# Autodesk Inventor assembly: VER2.0_MIR_CPY_MIR_MIR
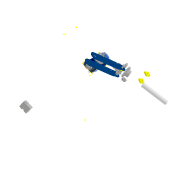
[picture p0: Inventor's stored thumbnail of the model, 180x180]
Saved by Autodesk Inventor 2020.5 (Build 245400000, 400)
## iProperties
Created: 2022-10-31
Part Number: VER2.0_MIR_CPY_MIR_MIR
Document SubType Name: Assembly
Designer: Administrator
Author: Administrator
## Documents named in this file (18)
- C:\Users\Administrator\Documents\kamuy2\kamuy2\VER2.0_MIR_CPY_MIR_MIR.iam
- C:\Users\Administrator\Documents\kamuy2\kamuy2\Parts\Part2_MIR_CPY_MIR_MIR.ipt
- C:\Users\Administrator\Documents\kamuy2\kamuy2\Parts\x-540_idle_MIR_CPY_MIR_MIR.ipt
- C:\Users\Administrator\Documents\kamuy2\kamuy2\Parts\GEABP1.0-32-10-A-12-KFC22-K3_Autodesk_Inventor_2020_20221101\AIS2020\GEABP1_0-32-10-A-12-KFC22-K3_MIR_CPY_MIR_MIR.iam
- C:\Users\Administrator\Documents\kamuy2\kamuy2\Parts\GEYK1.0-70-10-B-10K_Autodesk_Inventor_2020_20221114\AIS2020\GEYK1_0-70-10-B-10K_MIR_CPY_MIR_MIR.iam
- C:\Users\Administrator\Documents\kamuy2\kamuy2\Part16_MIR_CPY_MIR_MIR.ipt
- C:\Users\Administrator\Documents\kamuy2\kamuy2\Part1_MIR_CPY_MIR_MIR.ipt
- C:\Users\Administrator\Documents\kamuy2\kamuy2\Part13_MIR_CPY_MIR_MIR.ipt
- C:\Users\Administrator\Documents\kamuy2\kamuy2\Part17_MIR_CPY_MIR_MIR.ipt
- C:\Users\Administrator\Documents\kamuy2\kamuy2\Parts\SMYHF10_STEP_AP203AP214\SMYHF10_203_MIR_CPY_MIR_MIR.ipt
- C:\Users\Administrator\Documents\kamuy2\kamuy2\Parts\BGHK6800VV-30_Autodesk_Inventor_2020_20221102\AIS2020\BGHK6800VV-30_MIR_CPY_MIR_MIR.iam
- C:\Users\Administrator\Documents\kamuy2\kamuy2\Parts\XW540.N105.I101_MIR_CPY_MIR_MIR.ipt
- C:\Users\Administrator\Documents\kamuy2\kamuy2\Parts\NSFMKR10-67-KA22-A20_Autodesk_Inventor_2020_20221116\AIS2020\NSFMKR10-67-KA22-A20_MIR_CPY_MIR_MIR.iam
- C:\Users\Administrator\Documents\kamuy2\kamuy2\Parts\NSFMR10-37_Autodesk_Inventor_2020_20221116\AIS2020\NSFMR10-37(000_000)_MIR_CPY_MIR_MIR.iam
- C:\Users\Administrator\Documents\kamuy2\kamuy2\Parts\NSFMKRRA10-144-F3-S6-KA5-A18-KB108.5-B11_Autodesk_Inventor_2020_20221117\AIS2020\NSFMKRRA10-144-F3-S6-KA5-A18-KB108_5-B11_MIR_CPY_MIR_MIR.iam
- C:\Users\Administrator\Documents\kamuy2\kamuy2\LEG_MIR_MIR1_MIR.iam
- C:\Users\Administrator\Documents\kamuy2\kamuy2\Parts\BGTAB6900VV_Autodesk_Inventor_2020_20221121\AIS2020\BGTAB6900VV.iam
- C:\Users\Administrator\Documents\kamuy2\kamuy2\3dprinter\Part7.ipt
## Components (29 placed, 17 different names)
1. Part2_MIR_CPY_MIR_MIR:1
2. x-540_idle_MIR_CPY_MIR_MIR:1 — メイト:50, メイト:51, フラッシュ:58, フラッシュ:66, フラッシュ:68, メイト:258, メイト:154, メイト:166, フラッシュ:103, メイト:256
3. GEABP1_0-32-10-A-12-KFC22-K3_MIR_CPY_MIR_MIR:1 [sub-assembly] — メイト:50, メイト:51, フラッシュ:31
4. GEYK1_0-70-10-B-10K_MIR_CPY_MIR_MIR:1 [sub-assembly] — フラッシュ:61, メイト:248, フラッシュ:136
5. x-540_idle_MIR_CPY_MIR_MIR:2 — フラッシュ:58, フラッシュ:66, フラッシュ:68, メイト:85, メイト:86, メイト:168, フラッシュ:100, メイト:183, メイト:178, メイト:179, メイト:180
6. GEABP1_0-32-10-A-12-KFC22-K3_MIR_CPY_MIR_MIR:2 [sub-assembly] — メイト:85, メイト:86, フラッシュ:61
7. Part16_MIR_CPY_MIR_MIR:1 — メイト:258, フラッシュ:92, メイト:170
8. Part16_MIR_CPY_MIR_MIR:2 — フラッシュ:92, メイト:154, メイト:168, メイト:171, フラッシュ:141
9. Part1_MIR_CPY_MIR_MIR:1 — フラッシュ:100, メイト:171, フラッシュ:141
10. Part1_MIR_CPY_MIR_MIR:2 — メイト:166, メイト:170, メイト:183
11. Part13_MIR_CPY_MIR_MIR:1 — フラッシュ:103, メイト:172, フラッシュ:104, フラッシュ:108, メイト:208
12. Part17_MIR_CPY_MIR_MIR:1 — メイト:172, フラッシュ:104, フラッシュ:108, メイト:174, フラッシュ:105, メイト:177
13. SMYHF10_203_MIR_CPY_MIR_MIR:1 — メイト:174, フラッシュ:105, メイト:254
14. GEYK1_0-70-10-B-10K_MIR_CPY_MIR_MIR:2 [sub-assembly] — メイト:177, メイト:65, メイト:207
15. Part13_MIR_CPY_MIR_MIR:2 — メイト:178, メイト:179, メイト:180, メイト:194, フラッシュ:110, メイト:214
16. SMYHF10_203_MIR_CPY_MIR_MIR:2 — メイト:185, メイト:187, メイト:213
17. Part17_MIR_CPY_MIR_MIR:2 — メイト:185, メイト:187, メイト:194, フラッシュ:110, メイト:211, メイト:215, メイト:40
18. BGHK6800VV-30_MIR_CPY_MIR_MIR:1 [sub-assembly] — メイト:65, メイト:205, フラッシュ:32, フラッシュ:33, メイト:209, フラッシュ:115, フラッシュ:116
19. GEABP1_0-32-10-A-12-KFC22-K3_MIR_CPY_MIR_MIR:3 [sub-assembly] — メイト:203, メイト:204
20. XW540.N105.I101_MIR_CPY_MIR_MIR:1 — メイト:203, メイト:204, メイト:205, フラッシュ:32, フラッシュ:33, フラッシュ:17, メイト:42
21. NSFMKR10-67-KA22-A20_MIR_CPY_MIR_MIR:1 [sub-assembly] — メイト:207, メイト:208, メイト:209, メイト:254, メイト:41
22. BGHK6800VV-30_MIR_CPY_MIR_MIR:2 [sub-assembly] — フラッシュ:115, フラッシュ:116, メイト:211, メイト:212
23. NSFMR10-37(000_000)_MIR_CPY_MIR_MIR:1 [sub-assembly] — メイト:212, メイト:213, メイト:214, メイト:215, メイト:39
24. NSFMKRRA10-144-F3-S6-KA5-A18-KB108_5-B11_MIR_CPY_MIR_MIR:1 [sub-assembly] — メイト:248, フラッシュ:136, メイト:256, メイト:64
25. LEG_MIR_MIR1_MIR:1 [sub-assembly] — メイト:64, フラッシュ:31
26. BGTAB6900VV:1 [sub-assembly] — メイト:39, メイト:40, フラッシュ:18
27. BGTAB6900VV:2 [sub-assembly] — メイト:41, フラッシュ:17, メイト:42, フラッシュ:18
28. x-540_idle_MIR_CPY_MIR_MIR:3 — フラッシュ:19
29. Part7:1 — フラッシュ:19
## Relationships (61: Mate 42, Flush 19)
- メイト:50 [Mate] (4 mm): x-540_idle_MIR_CPY_MIR_MIR:1 ↔ GEABP1_0-32-10-A-12-KFC22-K3_MIR_CPY_MIR_MIR:1
- メイト:51 [Mate]: x-540_idle_MIR_CPY_MIR_MIR:1 ↔ GEABP1_0-32-10-A-12-KFC22-K3_MIR_CPY_MIR_MIR:1
- フラッシュ:58 [Flush]: x-540_idle_MIR_CPY_MIR_MIR:1 ↔ x-540_idle_MIR_CPY_MIR_MIR:2
- フラッシュ:66 [Flush]: x-540_idle_MIR_CPY_MIR_MIR:1 ↔ x-540_idle_MIR_CPY_MIR_MIR:2
- フラッシュ:68 [Flush]: x-540_idle_MIR_CPY_MIR_MIR:1 ↔ x-540_idle_MIR_CPY_MIR_MIR:2
- メイト:85 [Mate]: x-540_idle_MIR_CPY_MIR_MIR:2 ↔ GEABP1_0-32-10-A-12-KFC22-K3_MIR_CPY_MIR_MIR:2
- メイト:86 [Mate] (4 mm): x-540_idle_MIR_CPY_MIR_MIR:2 ↔ GEABP1_0-32-10-A-12-KFC22-K3_MIR_CPY_MIR_MIR:2
- フラッシュ:61 [Flush]: GEYK1_0-70-10-B-10K_MIR_CPY_MIR_MIR:1 ↔ GEABP1_0-32-10-A-12-KFC22-K3_MIR_CPY_MIR_MIR:2
- メイト:258 [Mate] (15.591 mm): x-540_idle_MIR_CPY_MIR_MIR:1 ↔ Part16_MIR_CPY_MIR_MIR:1
- フラッシュ:92 [Flush]: Part16_MIR_CPY_MIR_MIR:1 ↔ Part16_MIR_CPY_MIR_MIR:2
- メイト:154 [Mate] (15.591 mm): x-540_idle_MIR_CPY_MIR_MIR:1 ↔ Part16_MIR_CPY_MIR_MIR:2
- メイト:168 [Mate] (15.591 mm): x-540_idle_MIR_CPY_MIR_MIR:2 ↔ Part16_MIR_CPY_MIR_MIR:2
- フラッシュ:100 [Mate]: x-540_idle_MIR_CPY_MIR_MIR:2 ↔ Part1_MIR_CPY_MIR_MIR:1
- メイト:171 [Mate]: Part16_MIR_CPY_MIR_MIR:2 ↔ Part1_MIR_CPY_MIR_MIR:1
- フラッシュ:141 [Flush] (12.859 mm): Part16_MIR_CPY_MIR_MIR:2 ↔ Part1_MIR_CPY_MIR_MIR:1
- メイト:166 [Mate]: x-540_idle_MIR_CPY_MIR_MIR:1 ↔ Part1_MIR_CPY_MIR_MIR:2
- メイト:170 [Mate]: Part16_MIR_CPY_MIR_MIR:1 ↔ Part1_MIR_CPY_MIR_MIR:2
- メイト:183 [Mate]: x-540_idle_MIR_CPY_MIR_MIR:2 ↔ Part1_MIR_CPY_MIR_MIR:2
- フラッシュ:103 [Mate]: x-540_idle_MIR_CPY_MIR_MIR:1 ↔ Part13_MIR_CPY_MIR_MIR:1
- メイト:172 [Mate] (15 mm): Part13_MIR_CPY_MIR_MIR:1 ↔ Part17_MIR_CPY_MIR_MIR:1
- フラッシュ:104 [Flush]: Part13_MIR_CPY_MIR_MIR:1 ↔ Part17_MIR_CPY_MIR_MIR:1
- フラッシュ:108 [Flush]: Part13_MIR_CPY_MIR_MIR:1 ↔ Part17_MIR_CPY_MIR_MIR:1
- メイト:174 [Mate]: Part17_MIR_CPY_MIR_MIR:1 ↔ SMYHF10_203_MIR_CPY_MIR_MIR:1
- フラッシュ:105 [Flush] (0.1 mm): Part17_MIR_CPY_MIR_MIR:1 ↔ SMYHF10_203_MIR_CPY_MIR_MIR:1
- メイト:177 [Mate] (5 mm): Part17_MIR_CPY_MIR_MIR:1 ↔ GEYK1_0-70-10-B-10K_MIR_CPY_MIR_MIR:2
- メイト:178 [Mate]: x-540_idle_MIR_CPY_MIR_MIR:2 ↔ Part13_MIR_CPY_MIR_MIR:2
- メイト:179 [Mate]: x-540_idle_MIR_CPY_MIR_MIR:2 ↔ Part13_MIR_CPY_MIR_MIR:2
- メイト:180 [Mate]: x-540_idle_MIR_CPY_MIR_MIR:2 ↔ Part13_MIR_CPY_MIR_MIR:2
- メイト:185 [Mate]: SMYHF10_203_MIR_CPY_MIR_MIR:2 ↔ Part17_MIR_CPY_MIR_MIR:2
- メイト:187 [Mate]: SMYHF10_203_MIR_CPY_MIR_MIR:2 ↔ Part17_MIR_CPY_MIR_MIR:2
- メイト:194 [Mate] (15 mm): Part13_MIR_CPY_MIR_MIR:2 ↔ Part17_MIR_CPY_MIR_MIR:2
- フラッシュ:110 [Flush]: Part13_MIR_CPY_MIR_MIR:2 ↔ Part17_MIR_CPY_MIR_MIR:2
- メイト:65 [Mate] (4 mm): GEYK1_0-70-10-B-10K_MIR_CPY_MIR_MIR:2 ↔ BGHK6800VV-30_MIR_CPY_MIR_MIR:1
- メイト:203 [Mate]: GEABP1_0-32-10-A-12-KFC22-K3_MIR_CPY_MIR_MIR:3 ↔ XW540.N105.I101_MIR_CPY_MIR_MIR:1
- メイト:204 [Mate]: GEABP1_0-32-10-A-12-KFC22-K3_MIR_CPY_MIR_MIR:3 ↔ XW540.N105.I101_MIR_CPY_MIR_MIR:1
- メイト:205 [Mate] (6.591 mm): BGHK6800VV-30_MIR_CPY_MIR_MIR:1 ↔ XW540.N105.I101_MIR_CPY_MIR_MIR:1
- フラッシュ:32 [Flush]: BGHK6800VV-30_MIR_CPY_MIR_MIR:1 ↔ XW540.N105.I101_MIR_CPY_MIR_MIR:1
- フラッシュ:33 [Flush]: BGHK6800VV-30_MIR_CPY_MIR_MIR:1 ↔ XW540.N105.I101_MIR_CPY_MIR_MIR:1
- メイト:207 [Mate]: GEYK1_0-70-10-B-10K_MIR_CPY_MIR_MIR:2 ↔ NSFMKR10-67-KA22-A20_MIR_CPY_MIR_MIR:1
- メイト:208 [Mate]: Part13_MIR_CPY_MIR_MIR:1 ↔ NSFMKR10-67-KA22-A20_MIR_CPY_MIR_MIR:1
- メイト:209 [Mate]: BGHK6800VV-30_MIR_CPY_MIR_MIR:1 ↔ NSFMKR10-67-KA22-A20_MIR_CPY_MIR_MIR:1
- メイト:254 [Mate]: SMYHF10_203_MIR_CPY_MIR_MIR:1 ↔ NSFMKR10-67-KA22-A20_MIR_CPY_MIR_MIR:1
- フラッシュ:115 [Flush]: BGHK6800VV-30_MIR_CPY_MIR_MIR:1 ↔ BGHK6800VV-30_MIR_CPY_MIR_MIR:2
- フラッシュ:116 [Flush]: BGHK6800VV-30_MIR_CPY_MIR_MIR:1 ↔ BGHK6800VV-30_MIR_CPY_MIR_MIR:2
- メイト:211 [Mate] (4 mm): Part17_MIR_CPY_MIR_MIR:2 ↔ BGHK6800VV-30_MIR_CPY_MIR_MIR:2
- メイト:212 [Mate]: BGHK6800VV-30_MIR_CPY_MIR_MIR:2 ↔ NSFMR10-37(000_000)_MIR_CPY_MIR_MIR:1
- メイト:213 [Mate]: SMYHF10_203_MIR_CPY_MIR_MIR:2 ↔ NSFMR10-37(000_000)_MIR_CPY_MIR_MIR:1
- メイト:214 [Mate]: Part13_MIR_CPY_MIR_MIR:2 ↔ NSFMR10-37(000_000)_MIR_CPY_MIR_MIR:1
- メイト:215 [Mate]: Part17_MIR_CPY_MIR_MIR:2 ↔ NSFMR10-37(000_000)_MIR_CPY_MIR_MIR:1
- メイト:248 [Mate]: GEYK1_0-70-10-B-10K_MIR_CPY_MIR_MIR:1 ↔ NSFMKRRA10-144-F3-S6-KA5-A18-KB108_5-B11_MIR_CPY_MIR_MIR:1
- フラッシュ:136 [Flush] (-3 mm): GEYK1_0-70-10-B-10K_MIR_CPY_MIR_MIR:1 ↔ NSFMKRRA10-144-F3-S6-KA5-A18-KB108_5-B11_MIR_CPY_MIR_MIR:1
- メイト:256 [Mate] (31.591 mm): x-540_idle_MIR_CPY_MIR_MIR:1 ↔ NSFMKRRA10-144-F3-S6-KA5-A18-KB108_5-B11_MIR_CPY_MIR_MIR:1
- メイト:64 [Mate]: NSFMKRRA10-144-F3-S6-KA5-A18-KB108_5-B11_MIR_CPY_MIR_MIR:1 ↔ LEG_MIR_MIR1_MIR:1
- フラッシュ:31 [Flush]: GEABP1_0-32-10-A-12-KFC22-K3_MIR_CPY_MIR_MIR:1 ↔ LEG_MIR_MIR1_MIR:1
- メイト:39 [Mate]: NSFMR10-37(000_000)_MIR_CPY_MIR_MIR:1 ↔ BGTAB6900VV:1
- メイト:40 [Mate] (4 mm): Part17_MIR_CPY_MIR_MIR:2 ↔ BGTAB6900VV:1
- メイト:41 [Mate]: NSFMKR10-67-KA22-A20_MIR_CPY_MIR_MIR:1 ↔ BGTAB6900VV:2
- フラッシュ:17 [Flush]: XW540.N105.I101_MIR_CPY_MIR_MIR:1 ↔ BGTAB6900VV:2
- メイト:42 [Mate] (18.591 mm): XW540.N105.I101_MIR_CPY_MIR_MIR:1 ↔ BGTAB6900VV:2
- フラッシュ:18 [Flush]: BGTAB6900VV:1 ↔ BGTAB6900VV:2
- フラッシュ:19 [Flush]: x-540_idle_MIR_CPY_MIR_MIR:3 ↔ Part7:1
